# Autodesk Inventor assembly: ASY Кассета
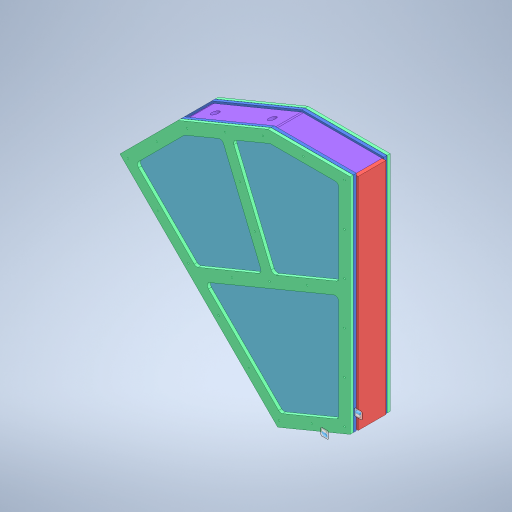
[picture p0: Inventor's stored thumbnail of the model, 512x512]
Saved by Autodesk Inventor 2024.2 (Build 282272000, 272)
## iProperties
Created: 2024-05-05
Part Number: ASY Кассета
Document SubType Name: Assembly
Designer: pokla
Author: pokla
## Documents named in this file (15)
- C:\Users\pokla\Documents\Inventor\ДФО\ДМФ\ДМФ 04.05.24 11-26\ASY Кассета.iam
- C:\Users\pokla\Documents\Inventor\ДФО\ДМФ\ДМФ 04.05.24 11-26\ДМС 201 Внешние рамки.ipt
- ДМС 201 Внешняя рамка.ipt
- C:\Users\pokla\Documents\Inventor\ДФО\ДМФ\ДМФ 04.05.24 11-26\ДМС 202 Верхний лист.ipt
- C:\Users\pokla\Documents\Inventor\ДФО\ДМФ\ДМФ 04.05.24 11-26\ДМС 203 Боковая часть.ipt
- C:\Users\pokla\Documents\Inventor\ДФО\ДМФ\ДМФ 04.05.24 11-26\ДМС 204 Нижний лист.ipt
- C:\Users\pokla\Documents\Inventor\ДФО\ДМФ\ДМФ 04.05.24 11-26\ДМС 205 Усилитель кассеты.ipt
- C:\Users\pokla\Documents\Inventor\ДФО\ДМФ\ДМФ 04.05.24 11-26\ДМС 206 Крепление сетки к кассете.ipt
- ДМС 206 Крепление сетки к кассете.ipt
- C:\Users\pokla\Documents\Inventor\ДФО\ДМФ\ДМФ 04.05.24 11-26\ДМС 207 Сетка кассеты.ipt
- ДМС 207 Сетка кассеты.ipt
- C:\Users\pokla\Documents\Inventor\ДФО\ДМФ\ДМФ 04.05.24 11-26\ДМС 201 Внешние рамки_MIR1.ipt
- C:\Users\pokla\Documents\Inventor\ДФО\ДМФ\ДМФ 04.05.24 11-26\ДМС 206 Крепление сетки к кассете_MIR1.ipt
- C:\Users\pokla\Documents\Inventor\ДФО\ДМФ\ДМФ 04.05.24 11-26\ДМС 207 Сетка кассеты_MIR1.ipt
- C:\Users\pokla\Documents\Inventor\ДФО\ДМФ\ДМФ 04.05.24 11-26\ДМС 208 Фиксатор расстояния кассет.ipt
## Components (12 placed, 11 different names)
1. ДМС 201 Внешняя рамка:1 — Rigid:1, Rigid:3, Rotational:1, Mate:2, Rigid:4, Rotational:2, Mate:3, Rigid:5, Rigid:8
2. ДМС 202 Верхний лист:1 — Rigid:3, Rigid:11
3. ДМС 203 Боковая часть:1 — Rotational:1, Mate:2
4. ДМС 204 Нижний лист:1 — Rigid:5, Mate:4
5. ДМС 205 Усилитель кассеты:1 — Rigid:8
6. ДМС 206 Крепление сетки к кассете:2 — Rigid:4
7. ДМС 207 Сетка кассеты:3 — Rigid:1
8. ДМС 203 Боковая часть:2 — Rotational:2, Mate:3
9. ДМС 201 Внешние рамки_MIR1:1 — Rigid:9, Rigid:10
10. ДМС 206 Крепление сетки к кассете_MIR1:1 — Rigid:9
11. ДМС 207 Сетка кассеты_MIR1:1 — Rigid:10
12. ДМС 208 Фиксатор расстояния кассет:1 — Rigid:11
## Relationships (13: WeldJoint 8, Mate 3, RevoluteJoint 2)
- Rigid:1 [WeldJoint]: ДМС 201 Внешняя рамка:1 ↔ ДМС 207 Сетка кассеты:3
- Rigid:3 [WeldJoint]: ДМС 201 Внешняя рамка:1 ↔ ДМС 202 Верхний лист:1
- Rotational:1 [RevoluteJoint]: ДМС 201 Внешняя рамка:1 ↔ ДМС 203 Боковая часть:1
- Mate:2: ДМС 201 Внешняя рамка:1 ↔ ДМС 203 Боковая часть:1
- Rigid:4 [WeldJoint] (0.5 mm): ДМС 201 Внешняя рамка:1 ↔ ДМС 206 Крепление сетки к кассете:2
- Rotational:2 [RevoluteJoint]: ДМС 201 Внешняя рамка:1 ↔ ДМС 203 Боковая часть:2
- Mate:3: ДМС 201 Внешняя рамка:1 ↔ ДМС 203 Боковая часть:2
- Rigid:5 [WeldJoint]: ДМС 201 Внешняя рамка:1 ↔ ДМС 204 Нижний лист:1
- Mate:4: ДМС 204 Нижний лист:1
- Rigid:8 [WeldJoint]: ДМС 201 Внешняя рамка:1 ↔ ДМС 205 Усилитель кассеты:1
- Rigid:9 [WeldJoint] (0.5 mm): ДМС 201 Внешние рамки_MIR1:1 ↔ ДМС 206 Крепление сетки к кассете_MIR1:1
- Rigid:10 [WeldJoint]: ДМС 201 Внешние рамки_MIR1:1 ↔ ДМС 207 Сетка кассеты_MIR1:1
- Rigid:11 [WeldJoint]: ДМС 202 Верхний лист:1 ↔ ДМС 208 Фиксатор расстояния кассет:1
